# Autodesk Inventor assembly: Combiner-Enclosure
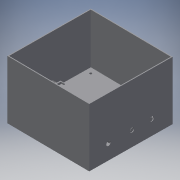
[picture p0: Inventor's stored thumbnail of the model, 180x180]
Saved by Autodesk Inventor 2018 (Build 220112000, 112)
## iProperties
Created: 2018-04-30
Part Number: Combiner-Enclosure
Document SubType Name: Assembly
Designer: bbramman
Author: bbramman
## Documents named in this file (4)
- C:\Users\bbramman\OneDrive\Documents\Trapped Ion Research (Grad)\Electronics\pll-evalboard-synthesizer\Box CAD\Combiner-Enclosure.iam
- C:\Users\bbramman\OneDrive\Documents\Trapped Ion Research (Grad)\Electronics\pll-evalboard-synthesizer\Box CAD\546-1550Z137-Combiner.ipt
- C:\Users\bbramman\OneDrive\Documents\Trapped Ion Research (Grad)\Electronics\pll-evalboard-synthesizer\Box CAD\3xCombiner.iam
- C:\Users\bbramman\OneDrive\Documents\Trapped Ion Research (Grad)\Electronics\pll-evalboard-synthesizer\Box CAD\Power-Reg.iam
## Components (3 placed, 3 different names)
1. 546-1550Z137-Combiner:1 — Insert:1, Insert:2
2. 3xCombiner:1 [sub-assembly] — Insert:2
3. Power-Reg:1 [sub-assembly] — Insert:1
## Relationships (2: Insert 2)
- Insert:1 (6.35 mm): 546-1550Z137-Combiner:1 ↔ Power-Reg:1
- Insert:2 (-21.59 mm): 546-1550Z137-Combiner:1 ↔ 3xCombiner:1
